# Autodesk Inventor assembly: ASY MSC Жабры
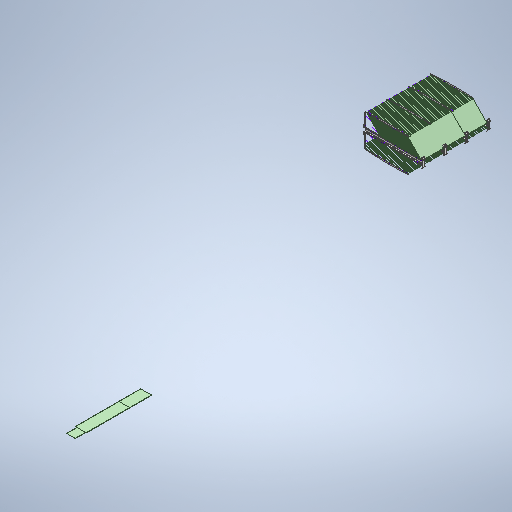
[picture p0: Inventor's stored thumbnail of the model, 512x512]
Saved by Autodesk Inventor 2025 (Build 290162010, 162A)
## iProperties
Created: 2024-08-31
Part Number: ASY MSC Жабры
Document SubType Name: Assembly
Designer: pokla
Author: pokla
## Documents named in this file (24)
- C:\Users\pokla\Documents\Inventor\Отстойник осветлитель\Manturovo_Se-clar-Gleb\ASY MSC Жабры.iam
- C:\Users\pokla\Documents\Inventor\Отстойник осветлитель\Manturovo_Se-clar-Gleb\MSC 0101 sheet gills.ipt
- C:\Users\pokla\Documents\Inventor\Отстойник осветлитель\Manturovo_Se-clar-Gleb\MSC 081 pillar 1.ipt
- C:\Users\pokla\Documents\Inventor\Отстойник осветлитель\Manturovo_Se-clar-Gleb\MSC 0102 sheet gills.ipt
- C:\Users\pokla\Documents\Inventor\Отстойник осветлитель\Manturovo_Se-clar-Gleb\MSC 0202 sheet gills.ipt
- C:\Users\pokla\Documents\Inventor\Отстойник осветлитель\Manturovo_Se-clar-Gleb\MSC 0103 sheet gills.ipt
- C:\Users\pokla\Documents\Inventor\Отстойник осветлитель\Manturovo_Se-clar-Gleb\MSC 0203 sheet gills.ipt
- C:\Users\pokla\Documents\Inventor\Отстойник осветлитель\Manturovo_Se-clar-Gleb\MSC 0104 sheet gills.ipt
- C:\Users\pokla\Documents\Inventor\Отстойник осветлитель\Manturovo_Se-clar-Gleb\MSC 0204 sheet gills.ipt
- C:\Users\pokla\Documents\Inventor\Отстойник осветлитель\Manturovo_Se-clar-Gleb\MSC 0105 sheet gills.ipt
- C:\Users\pokla\Documents\Inventor\Отстойник осветлитель\Manturovo_Se-clar-Gleb\MSC 0205 sheet gills.ipt
- C:\Users\pokla\Documents\Inventor\Отстойник осветлитель\Manturovo_Se-clar-Gleb\MSC 0106 sheet gills.ipt
- C:\Users\pokla\Documents\Inventor\Отстойник осветлитель\Manturovo_Se-clar-Gleb\MSC 0206 sheet gills.ipt
- C:\Users\pokla\Documents\Inventor\Отстойник осветлитель\Manturovo_Se-clar-Gleb\MSC 0107 sheet gills.ipt
- C:\Users\pokla\Documents\Inventor\Отстойник осветлитель\Manturovo_Se-clar-Gleb\MSC 0207 sheet gills.ipt
- C:\Users\pokla\Documents\Inventor\Отстойник осветлитель\Manturovo_Se-clar-Gleb\MSC 079 creen pillar.ipt
- C:\Users\pokla\Documents\Inventor\Отстойник осветлитель\Manturovo_Se-clar-Gleb\MSC DIM 085 tube belly.ipt
- C:\Users\pokla\Documents\Inventor\Отстойник осветлитель\Manturovo_Se-clar-Gleb\MSC 081 pillar 1_CPY.ipt
- C:\Users\pokla\Documents\Inventor\Отстойник осветлитель\Manturovo_Se-clar-Gleb\MSC 0211 string for sheets.ipt
- C:\Users\pokla\Documents\Inventor\Отстойник осветлитель\Manturovo_Se-clar-Gleb\MSC 079 top pillar.ipt
- C:\Users\pokla\Documents\Inventor\Отстойник осветлитель\Manturovo_Se-clar-Gleb\MSC DIM 085.1 heel.ipt
- C:\Users\pokla\Documents\Inventor\Отстойник осветлитель\Manturovo_Se-clar-Gleb\MSC 0201 sheet gills.ipt
- C:\Users\pokla\Documents\Inventor\Отстойник осветлитель\Manturovo_Se-clar-Gleb\MSC 0101 sheet gills_MIR.ipt
- C:\Users\pokla\Documents\Inventor\Отстойник осветлитель\Manturovo_Se-clar-Gleb\MSC 0201 sheet gills_MIR.ipt
## Components (332 placed, 24 different names)
1. MSC 0102 sheet gills:1 — Flush:12, Tangent:4, Tangent:5, Tangent:6, Mate:18, Flush:14, Flush:15
2. MSC 0202 sheet gills:1 — Mate:18, Flush:14, Flush:15
3. MSC 0103 sheet gills:1 — Flush:13, Tangent:7, Tangent:8, Tangent:9, Mate:19, Flush:16, Flush:17
4. MSC 0203 sheet gills:1 — Mate:19, Flush:16, Flush:17
5. MSC 0104 sheet gills:1 — Flush:18, Mate:20, Flush:19, Flush:20, Tangent:10, Tangent:11, Tangent:14
6. MSC 0204 sheet gills:1 — Mate:20, Flush:19, Flush:20
7. MSC 0105 sheet gills:1 — Mate:22, Flush:21, Flush:22, Flush:23, Tangent:12, Tangent:13, Tangent:15
8. MSC 0205 sheet gills:1 — Mate:22, Flush:21, Flush:22
9. MSC 0106 sheet gills:1 — Rigid:21
10. MSC 0206 sheet gills:1 — Rigid:21
11. MSC 0107 sheet gills:1 — Rigid:22
12. MSC 0207 sheet gills:1 — Rigid:22
13. MSC 079 creen pillar:1 — Rigid:11, Rigid:12, Flush:12, Flush:13, Flush:18, Flush:23
14. MSC 081 pillar 1_CPY:1 — Rigid:8, Rigid:9
15. MSC 079 top pillar:1 — Rigid:8, Rigid:11, Rigid:23
16. MSC 079 top pillar:2 — Rigid:9, Rigid:10, Rigid:24
17. MSC 079 creen pillar:2 — Rigid:10, Rigid:15
18. MSC 081 pillar 1:1 — Mate:11, Mate:12, Mate:13, Rigid:13, Rigid:16, Flush:6
19. MSC DIM 085 tube belly:1 — Rigid:6, Rigid:7, Mate:11, Mate:12, Mate:13, Mate:15, Mate:16, Flush:9
20. MSC DIM 085.1 heel:1 — Rigid:7
21. MSC DIM 085.1 heel:2 — Rigid:6
22. MSC 079 creen pillar:3
23. MSC 081 pillar 1_CPY:2
24. MSC 079 top pillar:3
25. MSC 079 top pillar:4
26. MSC 079 creen pillar:4
27. MSC 081 pillar 1:2
28. MSC DIM 085 tube belly:2
29. MSC DIM 085.1 heel:3
30. MSC DIM 085.1 heel:4
31. MSC 079 creen pillar:5
32. MSC 081 pillar 1_CPY:3
33. MSC 079 top pillar:5
34. MSC 079 top pillar:6
35. MSC 079 creen pillar:6
36. MSC 081 pillar 1:3
37. MSC DIM 085 tube belly:3
38. MSC DIM 085.1 heel:5
39. MSC DIM 085.1 heel:6
40. MSC 079 creen pillar:7
41. MSC 081 pillar 1_CPY:4
42. MSC 079 top pillar:7
43. MSC 079 top pillar:8
44. MSC 079 creen pillar:8
45. MSC 081 pillar 1:4
46. MSC DIM 085 tube belly:4
47. MSC DIM 085.1 heel:7
48. MSC DIM 085.1 heel:8
49. MSC 0211 string for sheets:4 — Rigid:15
50. MSC 0211 string for sheets:2 — Rigid:12, Tangent:1, Tangent:2
51. MSC 0211 string for sheets:5
52. MSC 0211 string for sheets:6
53. MSC 0211 string for sheets:7
54. MSC 0211 string for sheets:8
55. MSC 0211 string for sheets:9
56. MSC 0211 string for sheets:10
57. MSC 0211 string for sheets:11
58. MSC 0211 string for sheets:12
59. MSC 0211 string for sheets:13
60. MSC 0211 string for sheets:14
61. MSC 0211 string for sheets:15
62. MSC 0211 string for sheets:16
63. MSC 0211 string for sheets:17
64. MSC 0211 string for sheets:18
65. MSC 0211 string for sheets:19
66. MSC 0211 string for sheets:20
67. MSC 0211 string for sheets:21
68. MSC 0211 string for sheets:22
69. MSC 0211 string for sheets:23
70. MSC 0211 string for sheets:24
71. MSC 0211 string for sheets:25
72. MSC 0211 string for sheets:26
73. MSC 0211 string for sheets:27
74. MSC 0211 string for sheets:28
75. MSC 0211 string for sheets:29
76. MSC 0211 string for sheets:30
77. MSC 0211 string for sheets:31
78. MSC 0211 string for sheets:32
79. MSC 0211 string for sheets:33
80. MSC 0211 string for sheets:34
81. MSC 0211 string for sheets:35
82. MSC 0211 string for sheets:36
83. MSC 0211 string for sheets:37
84. MSC 0211 string for sheets:38
85. MSC 0211 string for sheets:39
86. MSC 0211 string for sheets:40
87. MSC 0211 string for sheets:41
88. MSC 0211 string for sheets:42
89. MSC 0211 string for sheets:43
90. MSC 0211 string for sheets:44
91. MSC 0211 string for sheets:45
92. MSC 0211 string for sheets:46
93. MSC 0211 string for sheets:47
94. MSC 0211 string for sheets:48
95. MSC 0211 string for sheets:49
96. MSC 0211 string for sheets:50
97. MSC 0211 string for sheets:51
98. MSC 0211 string for sheets:52
99. MSC 0211 string for sheets:53
100. MSC 0211 string for sheets:54
101. MSC 0211 string for sheets:55
102. MSC 0211 string for sheets:56
103. MSC 0211 string for sheets:57
104. MSC 0211 string for sheets:58
105. MSC 0211 string for sheets:59
106. MSC 0211 string for sheets:60
107. MSC 0211 string for sheets:61
108. MSC 0211 string for sheets:62
109. MSC 0211 string for sheets:63
110. MSC 0211 string for sheets:64
111. MSC 0211 string for sheets:3 — Rigid:16
112. MSC 0211 string for sheets:1 — Rigid:13, Tangent:3
113. MSC 0211 string for sheets:65
114. MSC 0211 string for sheets:66
115. MSC 0211 string for sheets:67
116. MSC 0211 string for sheets:68
117. MSC 0211 string for sheets:69
118. MSC 0211 string for sheets:70
119. MSC 0211 string for sheets:71
120. MSC 0211 string for sheets:72
121. MSC 0211 string for sheets:73
122. MSC 0211 string for sheets:74
123. MSC 0211 string for sheets:75
124. MSC 0211 string for sheets:76
125. MSC 0211 string for sheets:77
126. MSC 0211 string for sheets:78
127. MSC 0211 string for sheets:79
128. MSC 0211 string for sheets:80
129. MSC 0211 string for sheets:81
130. MSC 0211 string for sheets:82
131. MSC 0211 string for sheets:83
132. MSC 0211 string for sheets:84
133. MSC 0211 string for sheets:85
134. MSC 0211 string for sheets:86
135. MSC 0211 string for sheets:87
136. MSC 0211 string for sheets:88
137. MSC 0211 string for sheets:89
138. MSC 0211 string for sheets:90
139. MSC 0211 string for sheets:91
140. MSC 0211 string for sheets:92
141. MSC 0211 string for sheets:93
142. MSC 0211 string for sheets:94
143. MSC 0211 string for sheets:95
144. MSC 0211 string for sheets:96
145. MSC 0211 string for sheets:97
146. MSC 0211 string for sheets:98
147. MSC 0211 string for sheets:99
148. MSC 0211 string for sheets:100
149. MSC 0211 string for sheets:101
150. MSC 0211 string for sheets:102
151. MSC 0211 string for sheets:103
152. MSC 0211 string for sheets:104
153. MSC 0211 string for sheets:105
154. MSC 0211 string for sheets:106
155. MSC 0211 string for sheets:107
156. MSC 0211 string for sheets:108
157. MSC 0211 string for sheets:109
158. MSC 0211 string for sheets:110
159. MSC 0211 string for sheets:111
160. MSC 0211 string for sheets:112
161. MSC 0211 string for sheets:113
162. MSC 0211 string for sheets:114
163. MSC 0211 string for sheets:115
164. MSC 0211 string for sheets:116
165. MSC 0211 string for sheets:117
166. MSC 0211 string for sheets:118
167. MSC 0211 string for sheets:119
168. MSC 0211 string for sheets:120
169. MSC 0211 string for sheets:121
170. MSC 0211 string for sheets:122
171. MSC 0211 string for sheets:123
172. MSC 0211 string for sheets:124
173. MSC 0211 string for sheets:125
174. MSC 0211 string for sheets:126 — Tangent:6
175. MSC 0211 string for sheets:127
176. MSC 0211 string for sheets:128 — Tangent:9
177. MSC 0211 string for sheets:129
178. MSC 0211 string for sheets:130 — Tangent:14
179. MSC 0211 string for sheets:131
180. MSC 0211 string for sheets:132 — Tangent:15
181. MSC 0211 string for sheets:133
182. MSC 0211 string for sheets:134
183. MSC 0211 string for sheets:135
184. MSC 0211 string for sheets:136
185. MSC 0211 string for sheets:137
186. MSC 0211 string for sheets:138
187. MSC 0211 string for sheets:139
188. MSC 0211 string for sheets:140
189. MSC 0211 string for sheets:141
190. MSC 0211 string for sheets:142
191. MSC 0101 sheet gills.ipt:1 — Tangent:1, Tangent:2, Tangent:3, Flush:6, Flush:7, Flush:8, Mate:14
192. MSC 0201 sheet gills:1 — Flush:7, Flush:8, Mate:14
193. MSC 0101 sheet gills_MIR:1 — Mate:17, Flush:10, Flush:11
194. MSC 0201 sheet gills_MIR:1 — Mate:17, Flush:10, Flush:11
195. MSC 0101 sheet gills:2
196. MSC 0201 sheet gills:2
197. MSC 0101 sheet gills_MIR:2
198. MSC 0201 sheet gills_MIR:2
199. MSC 0101 sheet gills:3
200. MSC 0201 sheet gills:3
201. MSC 0101 sheet gills_MIR:3
202. MSC 0201 sheet gills_MIR:3
203. MSC 0101 sheet gills:4
204. MSC 0201 sheet gills:4
205. MSC 0101 sheet gills_MIR:4
206. MSC 0201 sheet gills_MIR:4
207. MSC 0101 sheet gills:5
208. MSC 0201 sheet gills:5
209. MSC 0101 sheet gills_MIR:5
210. MSC 0201 sheet gills_MIR:5
211. MSC 0101 sheet gills:6
212. MSC 0201 sheet gills:6
213. MSC 0101 sheet gills_MIR:6
214. MSC 0201 sheet gills_MIR:6
215. MSC 0101 sheet gills:7
216. MSC 0201 sheet gills:7
217. MSC 0101 sheet gills_MIR:7
218. MSC 0201 sheet gills_MIR:7
219. MSC 0101 sheet gills:8
220. MSC 0201 sheet gills:8
221. MSC 0101 sheet gills_MIR:8
222. MSC 0201 sheet gills_MIR:8
223. MSC 0101 sheet gills:9
224. MSC 0201 sheet gills:9
225. MSC 0101 sheet gills_MIR:9
226. MSC 0201 sheet gills_MIR:9
227. MSC 0101 sheet gills:10
228. MSC 0201 sheet gills:10
229. MSC 0101 sheet gills_MIR:10
230. MSC 0201 sheet gills_MIR:10
231. MSC 0101 sheet gills:11
232. MSC 0201 sheet gills:11
233. MSC 0101 sheet gills_MIR:11
234. MSC 0201 sheet gills_MIR:11
235. MSC 0101 sheet gills:12
236. MSC 0201 sheet gills:12
237. MSC 0101 sheet gills_MIR:12
238. MSC 0201 sheet gills_MIR:12
239. MSC 0101 sheet gills:13
240. MSC 0201 sheet gills:13
241. MSC 0101 sheet gills_MIR:13
242. MSC 0201 sheet gills_MIR:13
243. MSC 0101 sheet gills:14
244. MSC 0201 sheet gills:14
245. MSC 0101 sheet gills_MIR:14
246. MSC 0201 sheet gills_MIR:14
247. MSC 0101 sheet gills:15
248. MSC 0201 sheet gills:15
249. MSC 0101 sheet gills_MIR:15
250. MSC 0201 sheet gills_MIR:15
251. MSC 0101 sheet gills:16
252. MSC 0201 sheet gills:16
253. MSC 0101 sheet gills_MIR:16
254. MSC 0201 sheet gills_MIR:16
255. MSC 0101 sheet gills:17
256. MSC 0201 sheet gills:17
257. MSC 0101 sheet gills_MIR:17
258. MSC 0201 sheet gills_MIR:17
259. MSC 0101 sheet gills:18
260. MSC 0201 sheet gills:18
261. MSC 0101 sheet gills_MIR:18
262. MSC 0201 sheet gills_MIR:18
263. MSC 0101 sheet gills:19
264. MSC 0201 sheet gills:19
265. MSC 0101 sheet gills_MIR:19
266. MSC 0201 sheet gills_MIR:19
267. MSC 0101 sheet gills:20
268. MSC 0201 sheet gills:20
269. MSC 0101 sheet gills_MIR:20
270. MSC 0201 sheet gills_MIR:20
271. MSC 0101 sheet gills:21
272. MSC 0201 sheet gills:21
273. MSC 0101 sheet gills_MIR:21
274. MSC 0201 sheet gills_MIR:21
275. MSC 0101 sheet gills:22
276. MSC 0201 sheet gills:22
277. MSC 0101 sheet gills_MIR:22
278. MSC 0201 sheet gills_MIR:22
279. MSC 0101 sheet gills:23
280. MSC 0201 sheet gills:23
281. MSC 0101 sheet gills_MIR:23
282. MSC 0201 sheet gills_MIR:23
283. MSC 0101 sheet gills:24
284. MSC 0201 sheet gills:24
285. MSC 0101 sheet gills_MIR:24
286. MSC 0201 sheet gills_MIR:24
287. MSC 0101 sheet gills:25
288. MSC 0201 sheet gills:25
289. MSC 0101 sheet gills_MIR:25
290. MSC 0201 sheet gills_MIR:25
291. MSC 0101 sheet gills:26
292. MSC 0201 sheet gills:26
293. MSC 0101 sheet gills_MIR:26
294. MSC 0201 sheet gills_MIR:26
295. MSC 0101 sheet gills:27
296. MSC 0201 sheet gills:27
297. MSC 0101 sheet gills_MIR:27
298. MSC 0201 sheet gills_MIR:27
299. MSC 0101 sheet gills:28
300. MSC 0201 sheet gills:28
301. MSC 0101 sheet gills_MIR:28
302. MSC 0201 sheet gills_MIR:28
303. MSC 0101 sheet gills:29
304. MSC 0201 sheet gills:29
305. MSC 0101 sheet gills_MIR:29
306. MSC 0201 sheet gills_MIR:29
307. MSC 0101 sheet gills:30
308. MSC 0201 sheet gills:30
309. MSC 0101 sheet gills_MIR:30
310. MSC 0201 sheet gills_MIR:30
311. MSC 0101 sheet gills:31
312. MSC 0201 sheet gills:31
313. MSC 0101 sheet gills_MIR:31
314. MSC 0201 sheet gills_MIR:31
315. MSC 0211 string for sheets:143 — Rigid:23, Tangent:4, Tangent:5
316. MSC 0211 string for sheets:144 — Tangent:7, Tangent:8
317. MSC 0211 string for sheets:145 — Tangent:10, Tangent:11
318. MSC 0211 string for sheets:146 — Tangent:12, Tangent:13
319. MSC 0211 string for sheets:147
320. MSC 0211 string for sheets:148
321. MSC 0211 string for sheets:149
322. MSC 0211 string for sheets:150
323. MSC 0211 string for sheets:151
324. MSC 0211 string for sheets:152 — Rigid:24
325. MSC 0211 string for sheets:153
326. MSC 0211 string for sheets:154
327. MSC 0211 string for sheets:155
328. MSC 0211 string for sheets:156
329. MSC 0211 string for sheets:157
330. MSC 0211 string for sheets:158
331. MSC 0211 string for sheets:159
332. MSC 0211 string for sheets:160
## Component patterns: (4 elements, first: MSC 079 creen pillar:1 + MSC 081 pillar 1_CPY:1 + MSC 079 top pillar:1 + MSC 079 top pillar:2 + MSC 079 creen pillar:2 + MSC 081 pillar 1:1 + MSC DIM 085 tube belly:1 + MSC DIM 085.1 heel:1 + MSC DIM 085.1 heel:2), (31 elements, first: MSC 0211 string for sheets:4 + MSC 0211 string for sheets:2), (40 elements, first: MSC 0211 string for sheets:3 + MSC 0211 string for sheets:1), (31 elements, first: MSC 0101 sheet gills.ipt:1 + MSC 0201 sheet gills:1 + MSC 0101 sheet gills_MIR:1 + MSC 0201 sheet gills_MIR:1), (9 elements, first: MSC 0211 string for sheets:143), (9 elements, first: MSC 0211 string for sheets:152)
## Relationships (61: Flush 18, WeldJoint 15, Tangent 15, Mate 13)
- [Mate] (50 mm): MSC 0106 sheet gills:1 ↔ MSC 0107 sheet gills:1
- [WeldJoint]: MSC 081 pillar 1_CPY:1 ↔ MSC 081 pillar 1:1
- [Mate]: MSC 081 pillar 1_CPY:1 ↔ MSC 079 top pillar:1
- Rigid:6 [WeldJoint]: MSC DIM 085 tube belly:1 ↔ MSC DIM 085.1 heel:2
- Rigid:7 [WeldJoint]: MSC DIM 085 tube belly:1 ↔ MSC DIM 085.1 heel:1
- Mate:11: MSC 081 pillar 1:1 ↔ MSC DIM 085 tube belly:1
- Mate:12: MSC 081 pillar 1:1 ↔ MSC DIM 085 tube belly:1
- Mate:13: MSC 081 pillar 1:1 ↔ MSC DIM 085 tube belly:1
- Rigid:8 [WeldJoint]: MSC 081 pillar 1_CPY:1 ↔ MSC 079 top pillar:1
- Rigid:9 [WeldJoint]: MSC 081 pillar 1_CPY:1 ↔ MSC 079 top pillar:2
- Rigid:10 [WeldJoint]: MSC 079 top pillar:2 ↔ MSC 079 creen pillar:2
- Rigid:11 [WeldJoint]: MSC 079 creen pillar:1 ↔ MSC 079 top pillar:1
- Rigid:12 [WeldJoint] (-5 mm): MSC 079 creen pillar:1 ↔ MSC 0211 string for sheets:2
- Rigid:13 [WeldJoint] (-5 mm): MSC 081 pillar 1:1 ↔ MSC 0211 string for sheets:1
- Rigid:15 [WeldJoint] (-5 mm): MSC 079 creen pillar:2 ↔ MSC 0211 string for sheets:4
- Rigid:16 [WeldJoint] (-5 mm): MSC 081 pillar 1:1 ↔ MSC 0211 string for sheets:3
- Rigid:21 [WeldJoint]: MSC 0106 sheet gills:1 ↔ MSC 0206 sheet gills:1
- Rigid:22 [WeldJoint]: MSC 0107 sheet gills:1 ↔ MSC 0207 sheet gills:1
- Tangent:1: MSC 0211 string for sheets:2 ↔ MSC 0101 sheet gills.ipt:1
- Tangent:2: MSC 0211 string for sheets:2 ↔ MSC 0101 sheet gills.ipt:1
- Tangent:3: MSC 0211 string for sheets:1 ↔ MSC 0101 sheet gills.ipt:1
- Flush:6: MSC 081 pillar 1:1 ↔ MSC 0101 sheet gills.ipt:1
- Flush:7: MSC 0101 sheet gills.ipt:1 ↔ MSC 0201 sheet gills:1
- Flush:8: MSC 0101 sheet gills.ipt:1 ↔ MSC 0201 sheet gills:1
- Mate:14: MSC 0101 sheet gills.ipt:1 ↔ MSC 0201 sheet gills:1
- Mate:15: MSC DIM 085 tube belly:1
- Mate:16: MSC DIM 085 tube belly:1
- Flush:9: MSC DIM 085 tube belly:1
- Mate:17: MSC 0101 sheet gills_MIR:1 ↔ MSC 0201 sheet gills_MIR:1
- Flush:10: MSC 0101 sheet gills_MIR:1 ↔ MSC 0201 sheet gills_MIR:1
- Flush:11: MSC 0101 sheet gills_MIR:1 ↔ MSC 0201 sheet gills_MIR:1
- Rigid:23 [WeldJoint] (-5 mm): MSC 079 top pillar:1 ↔ MSC 0211 string for sheets:143
- Rigid:24 [WeldJoint] (-5 mm): MSC 079 top pillar:2 ↔ MSC 0211 string for sheets:152
- Flush:12: MSC 0102 sheet gills:1 ↔ MSC 079 creen pillar:1
- Tangent:4: MSC 0102 sheet gills:1 ↔ MSC 0211 string for sheets:143
- Tangent:5: MSC 0102 sheet gills:1 ↔ MSC 0211 string for sheets:143
- Tangent:6: MSC 0102 sheet gills:1 ↔ MSC 0211 string for sheets:126
- Flush:13: MSC 0103 sheet gills:1 ↔ MSC 079 creen pillar:1
- Tangent:7: MSC 0103 sheet gills:1 ↔ MSC 0211 string for sheets:144
- Tangent:8: MSC 0103 sheet gills:1 ↔ MSC 0211 string for sheets:144
- Tangent:9: MSC 0103 sheet gills:1 ↔ MSC 0211 string for sheets:128
- Mate:18: MSC 0102 sheet gills:1 ↔ MSC 0202 sheet gills:1
- Flush:14: MSC 0102 sheet gills:1 ↔ MSC 0202 sheet gills:1
- Flush:15: MSC 0102 sheet gills:1 ↔ MSC 0202 sheet gills:1
- Mate:19: MSC 0103 sheet gills:1 ↔ MSC 0203 sheet gills:1
- Flush:16: MSC 0103 sheet gills:1 ↔ MSC 0203 sheet gills:1
- Flush:17: MSC 0103 sheet gills:1 ↔ MSC 0203 sheet gills:1
- Flush:18: MSC 0104 sheet gills:1 ↔ MSC 079 creen pillar:1
- Mate:20: MSC 0104 sheet gills:1 ↔ MSC 0204 sheet gills:1
- Flush:19: MSC 0104 sheet gills:1 ↔ MSC 0204 sheet gills:1
- Flush:20: MSC 0104 sheet gills:1 ↔ MSC 0204 sheet gills:1
- Tangent:10: MSC 0104 sheet gills:1 ↔ MSC 0211 string for sheets:145
- Tangent:11: MSC 0104 sheet gills:1 ↔ MSC 0211 string for sheets:145
- Mate:22: MSC 0105 sheet gills:1 ↔ MSC 0205 sheet gills:1
- Flush:21: MSC 0105 sheet gills:1 ↔ MSC 0205 sheet gills:1
- Flush:22: MSC 0105 sheet gills:1 ↔ MSC 0205 sheet gills:1
- Flush:23: MSC 0105 sheet gills:1 ↔ MSC 079 creen pillar:1
- Tangent:12: MSC 0105 sheet gills:1 ↔ MSC 0211 string for sheets:146
- Tangent:13: MSC 0105 sheet gills:1 ↔ MSC 0211 string for sheets:146
- Tangent:14: MSC 0104 sheet gills:1 ↔ MSC 0211 string for sheets:130
- Tangent:15: MSC 0105 sheet gills:1 ↔ MSC 0211 string for sheets:132
